# Autodesk Inventor assembly: NewMechanumHubWithConnector
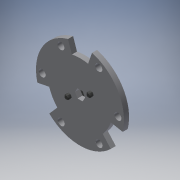
[picture p0: Inventor's stored thumbnail of the model, 180x180]
Saved by Autodesk Inventor 2017 (Build 210142000, 142)
## iProperties
Created: 2017-12-16
Part Number: NewMechanumHubWithConnector
Document SubType Name: Assembly
Designer: User
Author: User
## Documents named in this file (3)
- C:\Robotics\CAD\2017-18_CAD\Prototypes\NewMechanumHubWithConnector.iam
- C:\Robotics\CAD\2017-18_CAD\Prototypes\NewMechanumWheelHub.ipt
- C:\Robotics\CAD\COTSParts\Rev\REV-41-1147HexHub.ipt
## Components (2 placed, 2 different names)
1. NewMechanumWheelHub:1 — Mate:1, Mate:2, Mate:3
2. REV-41-1147HexHub:1 — Mate:1, Mate:2, Mate:3
## Relationships (3: Mate 3)
- Mate:1: NewMechanumWheelHub:1 ↔ REV-41-1147HexHub:1
- Mate:2: NewMechanumWheelHub:1 ↔ REV-41-1147HexHub:1
- Mate:3: NewMechanumWheelHub:1 ↔ REV-41-1147HexHub:1
